# Autodesk Inventor assembly: Montaje_motor_planetario_rueda
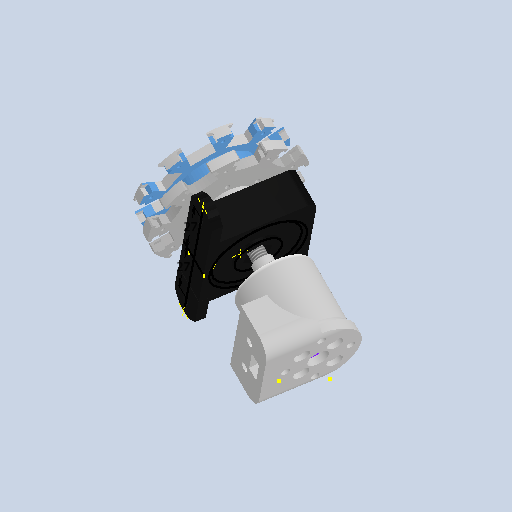
[picture p0: Inventor's stored thumbnail of the model, 512x512]
Saved by Autodesk Inventor 2024 (Build 280153000, 153)
## iProperties
Created: 2023-10-17
Part Number: Montaje_motor_planetario_rueda
Document SubType Name: Assembly
Designer: felip
Author: felip
## Documents named in this file (9)
- C:\Users\felip\Downloads\Piezas Planetario\Montaje_motor_planetario_rueda.iam
- C:\Users\felip\Downloads\Rueda 6cm\Rim_H6.ipt
- C:\Users\felip\Downloads\Rueda 6cm\Rim_6.ipt
- C:\Users\felip\Downloads\Piezas Planetario\planetary_gearbox_rueda_exterior_ipt2.ipt
- C:\Users\felip\Downloads\Piezas Planetario\output_wheel_ipt2.ipt
- C:\Users\felip\Downloads\Piezas Planetario\sun_gear_v2_ipt2.ipt
- C:\Users\felip\Downloads\Piezas Planetario\input_wheel_ipt2.ipt
- C:\Users\felip\Downloads\Piezas Planetario\bldc MOTOR.ipt
- C:\Users\felip\Downloads\SoporteV4.ipt
## Components (8 placed, 8 different names)
1. Rim_H6:1 — Rigid:1, Rotational:4
2. Rim_6:1 — Rigid:1
3. planetary_gearbox_rueda_exterior_ipt2:1 — Rotational:2, Rotational:3, Flush:1
4. output_wheel_ipt2:1 — Rotational:2
5. sun_gear_v2_ipt2:1 — Rotational:1, Rotational:3, Rotational:4, Rotational:5
6. input_wheel_ipt2:1 — Rotational:1
7. bldc MOTOR:1 — Rotational:5, Rotational:6
8. SoporteV4:1 — Flush:1, Rotational:6
## Relationships (8: RevoluteJoint 6, WeldJoint 1, Flush 1)
- Rigid:1 [WeldJoint]: Rim_H6:1 ↔ Rim_6:1
- Rotational:1 [RevoluteJoint] (1 mm): sun_gear_v2_ipt2:1 ↔ input_wheel_ipt2:1
- Rotational:2 [RevoluteJoint] (-1.8 mm): planetary_gearbox_rueda_exterior_ipt2:1 ↔ output_wheel_ipt2:1
- Rotational:3 [RevoluteJoint]: planetary_gearbox_rueda_exterior_ipt2:1 ↔ sun_gear_v2_ipt2:1
- Rotational:4 [RevoluteJoint] (3 mm): Rim_H6:1 ↔ sun_gear_v2_ipt2:1
- Rotational:5 [RevoluteJoint] (-4.4 mm): sun_gear_v2_ipt2:1 ↔ bldc MOTOR:1
- Flush:1 (-0.5 mm): planetary_gearbox_rueda_exterior_ipt2:1 ↔ SoporteV4:1
- Rotational:6 [RevoluteJoint]: bldc MOTOR:1 ↔ SoporteV4:1
